# Autodesk Inventor assembly: CartesianRobotWorkSpace
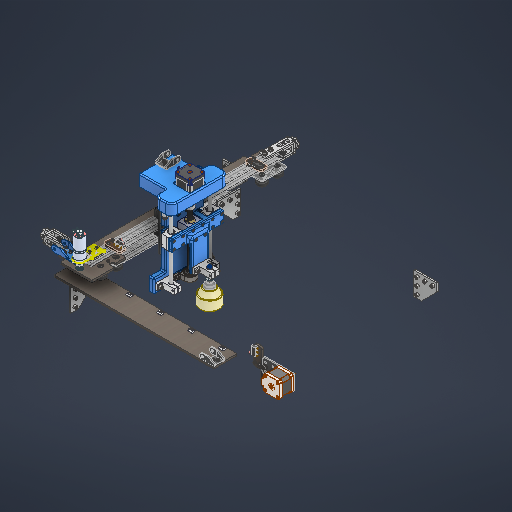
[picture p0: Inventor's stored thumbnail of the model, 512x512]
Saved by Autodesk Inventor 2027.1 (Build 311270010, 270A)
## iProperties
Created: 2026-09-29
Part Number: CartesianRobotWorkSpace
Document SubType Name: Assembly
Designer: SDS Scholar
Author: SDS Scholar
## Documents named in this file (40)
- E:\Apps\AutodeskInventor\University\MCT333_Design_of_Mechatronics_Systems_1\CAD\cartesian_robot_workspace\CartesianRobotWorkSpace.iam
- E:\Apps\AutodeskInventor\University\MCT333_Design_of_Mechatronics_Systems_1\CAD\off_the_shelf_components\AluminiumExtrusion\AluminiumExtrusion2020\Pillars.ipt
- E:\Apps\AutodeskInventor\University\MCT333_Design_of_Mechatronics_Systems_1\CAD\off_the_shelf_components\CornerBracket2020\CornerBracket2020.ipt
- E:\Apps\AutodeskInventor\University\MCT333_Design_of_Mechatronics_Systems_1\CAD\en-US\en-US\SS-ISO 4762\ISO 4762 - M5 x 10SS-ISO.ipt
- E:\Apps\AutodeskInventor\University\MCT333_Design_of_Mechatronics_Systems_1\CAD\off_the_shelf_components\T_nuts\Slider T-Nut for 2020 - M5.ipt
- E:\Apps\AutodeskInventor\University\MCT333_Design_of_Mechatronics_Systems_1\CAD\off_the_shelf_components\RightAngleCornerPlate2020\2020 corner joining plate v1.ipt
- E:\Apps\AutodeskInventor\University\MCT333_Design_of_Mechatronics_Systems_1\CAD\off_the_shelf_components\AluminiumExtrusion\Extrusion2040\2040extrusion_ipt\X_Axis.ipt
- E:\Apps\AutodeskInventor\University\MCT333_Design_of_Mechatronics_Systems_1\CAD\off_the_shelf_components\AluminiumExtrusion\AluminiumExtrusion2020\SupportBeam.ipt
- E:\Apps\AutodeskInventor\University\MCT333_Design_of_Mechatronics_Systems_1\CAD\off_the_shelf_components\VSoltGantrySetAllSizes\20mm Gantry Set\20mm Gantry Set.ipt
- E:\Apps\AutodeskInventor\University\MCT333_Design_of_Mechatronics_Systems_1\CAD\off_the_shelf_components\RightAngleCornerPlate2020\2020 corner joining plate v1_MIR2.ipt
- E:\Apps\AutodeskInventor\University\MCT333_Design_of_Mechatronics_Systems_1\CAD\off_the_shelf_components\T_nuts\Slider T-Nut for 2020 - M5_MIR2.ipt
- E:\Apps\AutodeskInventor\University\MCT333_Design_of_Mechatronics_Systems_1\CAD\off_the_shelf_components\nema-17-23-stepper-motor-mounts\NEMA 17 Flat.ipt
- E:\Apps\AutodeskInventor\University\MCT333_Design_of_Mechatronics_Systems_1\CAD\off_the_shelf_components\GT2BeltTensioner\2020 Belt Tensioner G_K.ipt
- E:\Apps\AutodeskInventor\University\MCT333_Design_of_Mechatronics_Systems_1\CAD\cartesian_robot_workspace\Y_Axis.iam
- E:\Apps\AutodeskInventor\University\MCT333_Design_of_Mechatronics_Systems_1\CAD\cartesian_robot_workspace\Z Axis\Z-Axis.iam
- E:\Apps\AutodeskInventor\University\MCT333_Design_of_Mechatronics_Systems_1\CAD\motors_and_actuators\nema17_stepper_motor\Nema17\Nema17.ipt
- E:\Apps\AutodeskInventor\University\MCT333_Design_of_Mechatronics_Systems_1\CAD\off_the_shelf_components\gt2_pulley_6\GT2 Pulley Assembly With Grub Screws\GT2 Pulley Assembly With Grub Screws.ipt
- E:\Apps\AutodeskInventor\University\MCT333_Design_of_Mechatronics_Systems_1\CAD\cartesian_robot_workspace\Z_Axis_1\Z-Axis.iam
- E:\Apps\AutodeskInventor\University\MCT333_Design_of_Mechatronics_Systems_1\CAD\cartesian_robot_workspace\LimitSwitchMountPlate.ipt
- E:\Apps\AutodeskInventor\University\MCT333_Design_of_Mechatronics_Systems_1\CAD\cartesian_robot_workspace\Z_Axis_1\NO-NC Bump Switch\NO-NC Bump Switch.ipt
- E:\Apps\AutodeskInventor\University\MCT333_Design_of_Mechatronics_Systems_1\CAD\cartesian_robot_workspace\Z_Axis_1\Slider T-Nut for 2020 - M3.ipt
- C:\Users\SDS Scholar\Documents\Inventor\Content Center Files\R2027\en-US\ISO 4762(2)\ISO 4762 - M3 x 10ISO.ipt
- C:\Users\SDS Scholar\Documents\Inventor\Content Center Files\R2027\en-US\ANSI B18.22 M\ANSI B18.22M - 3 N.ipt
- E:\Apps\AutodeskInventor\University\MCT333_Design_of_Mechatronics_Systems_1\CAD\cartesian_robot_workspace\Z_Axis_1\2020 Belt Tensioner G_K.ipt
- E:\Apps\AutodeskInventor\University\MCT333_Design_of_Mechatronics_Systems_1\CAD\cartesian_robot_workspace\Z_Axis_1\M4 T slot nut - 2020\M4 T slot nut - 2020.ipt
- C:\Users\SDS Scholar\Documents\Inventor\Content Center Files\R2027\en-US\ISO 4762(2)\ISO 4762 - M4 x 12ISO.ipt
- C:\Users\SDS Scholar\Documents\Inventor\Content Center Files\R2027\en-US\ANSI B18.22 M\ANSI B18.22M - 4 N.ipt
- E:\Apps\AutodeskInventor\University\MCT333_Design_of_Mechatronics_Systems_1\CAD\Drag Chain Support (Y Axis).ipt
- E:\Apps\AutodeskInventor\University\MCT333_Design_of_Mechatronics_Systems_1\CAD\cartesian_robot_workspace\Z_Axis_1\Drag Chain Start Link.ipt
- C:\Users\SDS Scholar\Documents\Inventor\Content Center Files\R2027\en-US\ANSI B18.22 M\ANSI B18.22M - 5 N.ipt
- C:\Users\SDS Scholar\Documents\Inventor\Content Center Files\R2027\en-US\SS-ISO 4762\ISO 4762 - M5 x 12SS-ISO.ipt
- E:\Apps\AutodeskInventor\University\MCT333_Design_of_Mechatronics_Systems_1\CAD\cartesian_robot_workspace\Z_Axis_1\LimitSwitchMountPlate (X Axis).ipt
- C:\Users\SDS Scholar\Documents\Inventor\Content Center Files\R2027\en-US\ISO 4762(2)\ISO 4762 - M3 x 12ISO.ipt
- E:\Apps\AutodeskInventor\University\MCT333_Design_of_Mechatronics_Systems_1\CAD\en-US\en-US\ISO 4762(2)\ISO 4762 - M2 x 16ISO.ipt
- E:\Apps\AutodeskInventor\University\MCT333_Design_of_Mechatronics_Systems_1\CAD\en-US\en-US\ISO 4032(2)\ISO 4032 - M2 - ISO.ipt
- E:\Apps\AutodeskInventor\University\MCT333_Design_of_Mechatronics_Systems_1\CAD\en-US\en-US\Plain Washer Metric\ANSI B18.22M - 2 N.ipt
- E:\Apps\AutodeskInventor\University\MCT333_Design_of_Mechatronics_Systems_1\CAD\en-US\en-US\ISO 7046-1 Z(1)\ISO 7045 - M2.5 x 12_ - 4.8 - Z - ISO.ipt
- E:\Apps\AutodeskInventor\University\MCT333_Design_of_Mechatronics_Systems_1\CAD\en-US\en-US\Plain Washer Metric\ANSI B18.22M - 2.5 N.ipt
- E:\Apps\AutodeskInventor\University\MCT333_Design_of_Mechatronics_Systems_1\CAD\en-US\en-US\ISO 4032(2)\ISO 4032 - M3 - ISO.ipt
- E:\Apps\AutodeskInventor\University\MCT333_Design_of_Mechatronics_Systems_1\CAD\DESIGN1_CAD_parameters.xlsx
## Components (190 placed, 36 different names)
1. Z-Axis:1 [sub-assembly] — Tangent:9, Tangent:10, Mate:231, Mate:232
2. Z-Axis:2 [sub-assembly] — Mate:299, Mate:300, Tangent:11, Flush:334, Mate:455, Mate:475
3. LimitSwitchMountPlate:1 — Mate:326, Mate:327, Mate:328, Flush:330
4. NO-NC Bump Switch:1
5. Slider T-Nut for 2020 - M3:1 — Mate:330, Angle:2, Flush:331
6. Slider T-Nut for 2020 - M3:2 — Mate:329, Angle:1, Flush:331, Mate:331
7. ISO 4762 M3 x 10:1 — Mate:327, Mate:330
8. ISO 4762 M3 x 10:2 — Mate:328, Mate:329
9. Plain Washer (Metric) 3 N:1
10. Plain Washer (Metric) 3 N:2
11. ISO 4762 M2 x 16:7
12. ISO 4032 M2:7
13. Plain Washer (Metric) 2 N:8
14. ISO 4762 M2 x 16:8
15. ISO 4032 M2:8
16. Plain Washer (Metric) 2 N:9
17. Drag Chain Start Link:1 — Mate:349, Mate:350, Mate:351, Flush:334, Mate:462, Mate:463, Mate:464, Mate:465
18. Drag Chain Support (Y Axis):1 — Mate:347, Flush:333, Mate:348, Mate:349, Mate:350, Mate:351, Mate:466, Mate:467, Mate:468, Mate:472, Mate:474
19. 2020 Belt Tensioner G_K:3 — Flush:336, Mate:382, Mate:383, Mate:455
20. M4 T slot nut - 2020:3 — Mate:384
21. M4 T slot nut - 2020:4
22. ISO 4762 M4 x 12:3
23. ISO 4762 M4 x 12:4
24. Plain Washer (Metric) 4 N:3
25. Plain Washer (Metric) 4 N:4
26. SS ISO 4762 M5 x 12:1 — Mate:385, Mate:387, Mate:393
27. SS ISO 4762 M5 x 12:2 — Mate:388, Mate:389
28. Slider T-Nut for 2020 - M5:52 — Flush:337, Flush:338, Mate:392, Angle:14
29. Slider T-Nut for 2020 - M5:53 — Flush:337, Angle:14
30. NEMA 17 Flat:2 — Mate:386, Mate:390, Mate:391, Angle:8, Angle:9, Mate:400, Mate:407, Mate:408, Mate:409, Mate:449
31. Nema17:2 — Mate:381, Angle:9, Mate:394, Mate:395, Mate:396, Mate:397
32. GT2 Pulley Assembly With Grub Screws:2 — Mate:381
33. Plain Washer (Metric) 5 N:1 — Mate:385, Mate:386, Mate:387
34. Plain Washer (Metric) 5 N:2 — Mate:388, Mate:389, Mate:390
35. ISO 7045 Z M2.5 x 12 - 4.8 - Z:6 — Mate:394, Mate:401, Mate:404
36. ISO 7045 Z M2.5 x 12 - 4.8 - Z:7 — Mate:395, Mate:398, Mate:399
37. ISO 7045 Z M2.5 x 12 - 4.8 - Z:8 — Mate:396, Mate:402, Mate:406
38. ISO 7045 Z M2.5 x 12 - 4.8 - Z:9 — Mate:397, Mate:403, Mate:405
39. Plain Washer (Metric) 2.5 N:6 — Mate:401, Mate:404, Mate:408
40. Plain Washer (Metric) 2.5 N:7 — Mate:403, Mate:405, Mate:409
41. Plain Washer (Metric) 2.5 N:8 — Mate:402, Mate:406, Mate:407
42. Plain Washer (Metric) 2.5 N:9 — Mate:398, Mate:399, Mate:400
43. Slider T-Nut for 2020 - M3:3 — Angle:12, Angle:13, Flush:339, Mate:447
44. Slider T-Nut for 2020 - M3:4 — Angle:13, Flush:339
45. ISO 4762 M3 x 10:3 — Mate:444, Mate:448
46. ISO 4762 M3 x 10:4 — Mate:443
47. Plain Washer (Metric) 3 N:3 — Mate:445
48. Plain Washer (Metric) 3 N:4 — Mate:446
49. LimitSwitchMountPlate (X Axis):1 — Angle:11, Mate:442, Mate:443, Mate:444, Mate:445, Mate:446, Angle:12, Mate:449, Mate:450, Mate:451, Mate:452, Mate:453, Mate:454, Mate:475
50. NO-NC Bump Switch:3 — Mate:452
51. ISO 4762 M2 x 16:9 — Mate:451
52. ISO 4032 M2:9 — Mate:454
53. Plain Washer (Metric) 2 N:10
54. ISO 4762 M2 x 16:10 — Mate:450
55. ISO 4032 M2:10 — Mate:453
56. Plain Washer (Metric) 2 N:11
57. ISO 4762 M3 x 12:1 — Mate:462, Mate:468
58. Plain Washer (Metric) 3 N:5 — Mate:463
59. ISO 4032 M3:3 — Mate:467
60. ISO 4762 M3 x 12:2 — Mate:464
61. Plain Washer (Metric) 3 N:6 — Mate:465
62. ISO 4032 M3:4 — Mate:466
63. SupportBeam:1 — Mate:123, Mate:124, Mate:125, Mate:126, Mate:138, Mate:141, Mate:143, Mate:202
64. X_Axis:1 — Mate:32, Mate:33, Mate:34, Mate:35, Mate:36, Mate:37, Mate:48, Mate:49, Mate:56, Mate:59, Flush:3, Tangent:1, Tangent:2, Mate:217, Mate:271, Mate:299, Tangent:11, Mate:326, Flush:330, Angle:1, Angle:2, Mate:331, Mate:347, Flush:333, Flush:336, Mate:382, Mate:383, Mate:384, Mate:391, Angle:8, Flush:338, Mate:392, Mate:393, Angle:11, Mate:442, Mate:447, Mate:448, Angle:15, Mate:473
65. X_Axis:2 — Mate:89, Mate:90, Mate:91, Mate:92, Mate:93, Mate:94, Mate:107, Mate:110, Mate:113, Mate:115, Flush:4, Tangent:5, Tangent:6, Mate:225, Mate:300
66. 2020 Belt Tensioner G_K:1 — Mate:271
67. 20mm Gantry Set:1 — Tangent:1, Tangent:2, Flush:5, Mate:171, Flush:9, Mate:229, Mate:230
68. 20mm Gantry Set:2 — Tangent:5, Tangent:6, Flush:5, Mate:174, Mate:177, Flush:8, Flush:9
69. Y_Axis:1 [sub-assembly] — Mate:167, Mate:168, Mate:169, Mate:170, Mate:173, Mate:176, Mate:177, Flush:8, Tangent:9, Tangent:10, Mate:231, Mate:232
70. Slider T-Nut for 2020 - M5:44 — Mate:167, Mate:168, Mate:172
71. Slider T-Nut for 2020 - M5:45 — Mate:169, Mate:170, Mate:175
72. SS ISO 4762 M5 x 10:62 — Mate:174, Mate:175, Mate:176
73. SS ISO 4762 M5 x 10:63 — Mate:171, Mate:172, Mate:173
74. Pillars:1 — Flush:10, Flush:11, Mate:183, Mate:184, Mate:185, Mate:186, Mate:187, Mate:188, Mate:189, Flush:191, Flush:192, Mate:190, Symmetry:1, Mate:191, Mate:192, Mate:193, Mate:194, Mate:195, Mate:196, Mate:197, Mate:198, Mate:199, Mate:200, Mate:201, Mate:202, Mate:476, Mate:477
75. SS ISO 4762 M5 x 10:2 — Mate:28, Mate:29, Mate:189
76. Slider T-Nut for 2020 - M5:2 — Mate:29, Mate:186, Mate:187
77. Slider T-Nut for 2020 - M5:1 — Mate:21, Mate:184, Mate:185
78. SS ISO 4762 M5 x 10:1 — Mate:20, Mate:21, Mate:31, Mate:188
79. CornerBracket2020:1 — Mate:20, Mate:31, Flush:191, Flush:340, Flush:341
80. CornerBracket2020:4 — Mate:28, Flush:192, Mate:190
81. CornerBracket2020:12 — Flush:341, Mate:477
82. CornerBracket2020:11 — Mate:476, Flush:340
83. Pillars:2 — Mate:218, Mate:219, Mate:220, Mate:221, Mate:222, Mate:223, Mate:224, Mate:225
84. SS ISO 4762 M5 x 10:64
85. Slider T-Nut for 2020 - M5:46
86. Slider T-Nut for 2020 - M5:47
87. SS ISO 4762 M5 x 10:65
88. CornerBracket2020:5
89. CornerBracket2020:6
90. CornerBracket2020:13
91. CornerBracket2020:14
92. Pillars:3 — Symmetry:1, Mate:348
93. SS ISO 4762 M5 x 10:66
94. Slider T-Nut for 2020 - M5:48
95. Slider T-Nut for 2020 - M5:49
96. SS ISO 4762 M5 x 10:67
97. CornerBracket2020:7
98. CornerBracket2020:8
99. CornerBracket2020:15
100. CornerBracket2020:16
101. Pillars:4 — Mate:210, Mate:211, Mate:212, Mate:213, Mate:214, Mate:215, Mate:216, Mate:217
102. SS ISO 4762 M5 x 10:68
103. Slider T-Nut for 2020 - M5:50
104. Slider T-Nut for 2020 - M5:51
105. SS ISO 4762 M5 x 10:69
106. CornerBracket2020:9
107. CornerBracket2020:10
108. CornerBracket2020:17
109. CornerBracket2020:18
110. Slider T-Nut for 2020 - M5:54 — Angle:15, Mate:473
111. Plain Washer (Metric) 5 N:3 — Mate:474
112. SS ISO 4762 M5 x 12:3 — Mate:472
113. Slider T-Nut for 2020 - M5:55
114. Plain Washer (Metric) 5 N:4
115. SS ISO 4762 M5 x 12:4
116. Slider T-Nut for 2020 - M5:56
117. Plain Washer (Metric) 5 N:5
118. SS ISO 4762 M5 x 12:5
119. Slider T-Nut for 2020 - M5:57
120. Plain Washer (Metric) 5 N:6
121. SS ISO 4762 M5 x 12:6
122. Slider T-Nut for 2020 - M5:58
123. Plain Washer (Metric) 5 N:7
124. SS ISO 4762 M5 x 12:7
125. 2020 corner joining plate v1:6 — Mate:127, Mate:130, Mate:133, Mate:136, Mate:139, Mate:143, Mate:144, Mate:201
126. Slider T-Nut for 2020 - M5:35 — Mate:131, Mate:192, Mate:195
127. Slider T-Nut for 2020 - M5:36 — Mate:123, Mate:124, Mate:137
128. Slider T-Nut for 2020 - M5:37 — Mate:134, Mate:191, Mate:194, Mate:196
129. Slider T-Nut for 2020 - M5:38 — Mate:125, Mate:126, Mate:140
130. Slider T-Nut for 2020 - M5:39 — Mate:128, Mate:193, Mate:197
131. SS ISO 4762 M5 x 10:48 — Mate:127, Mate:128, Mate:198
132. SS ISO 4762 M5 x 10:49 — Mate:139, Mate:140, Mate:141
133. SS ISO 4762 M5 x 10:50 — Mate:130, Mate:131, Mate:199
134. SS ISO 4762 M5 x 10:51 — Mate:133, Mate:134, Mate:200
135. SS ISO 4762 M5 x 10:52 — Mate:136, Mate:137, Mate:138
136. 2020 corner joining plate v1_MIR2:1
137. Slider T-Nut for 2020 - M5_MIR2:1
138. Slider T-Nut for 2020 - M5_MIR2:2
139. Slider T-Nut for 2020 - M5_MIR2:3
140. Slider T-Nut for 2020 - M5_MIR2:4
141. Slider T-Nut for 2020 - M5_MIR2:5
142. SS ISO 4762 M5 x 10:53
143. SS ISO 4762 M5 x 10:54
144. SS ISO 4762 M5 x 10:55
145. SS ISO 4762 M5 x 10:56
146. SS ISO 4762 M5 x 10:57
147. 2020 corner joining plate v1:1 — Mate:42, Mate:46, Mate:49, Mate:51, Mate:54, Mate:57, Flush:3, Mate:216, Mate:230
148. Slider T-Nut for 2020 - M5:9 — Mate:36, Mate:37, Mate:55
149. Slider T-Nut for 2020 - M5:10 — Mate:52, Mate:212, Mate:213
150. Slider T-Nut for 2020 - M5:11 — Mate:43, Mate:210, Mate:211
151. Slider T-Nut for 2020 - M5:12 — Mate:34, Mate:35, Mate:58
152. Slider T-Nut for 2020 - M5:13 — Mate:32, Mate:33, Mate:47
153. SS ISO 4762 M5 x 10:9 — Mate:42, Mate:43, Mate:215
154. SS ISO 4762 M5 x 10:10 — Mate:46, Mate:47, Mate:48
155. SS ISO 4762 M5 x 10:11 — Mate:54, Mate:55, Mate:56
156. SS ISO 4762 M5 x 10:12 — Mate:51, Mate:52, Mate:214
157. SS ISO 4762 M5 x 10:13 — Mate:57, Mate:58, Mate:59
158. 2020 corner joining plate v1:2 — Mate:229
159. Slider T-Nut for 2020 - M5:14
160. Slider T-Nut for 2020 - M5:15
161. Slider T-Nut for 2020 - M5:16
162. Slider T-Nut for 2020 - M5:17
163. Slider T-Nut for 2020 - M5:18
164. SS ISO 4762 M5 x 10:14
165. SS ISO 4762 M5 x 10:15
166. SS ISO 4762 M5 x 10:16
167. SS ISO 4762 M5 x 10:17
168. SS ISO 4762 M5 x 10:18
169. 2020 corner joining plate v1:4 — Mate:99, Mate:102, Mate:105, Mate:108, Mate:111, Mate:115, Flush:4, Mate:224
170. Slider T-Nut for 2020 - M5:25 — Mate:93, Mate:94, Mate:106
171. Slider T-Nut for 2020 - M5:26 — Mate:103, Mate:218, Mate:219
172. Slider T-Nut for 2020 - M5:27 — Mate:100, Mate:220, Mate:221
173. Slider T-Nut for 2020 - M5:28 — Mate:91, Mate:92, Mate:109
174. Slider T-Nut for 2020 - M5:29 — Mate:89, Mate:90, Mate:112
175. SS ISO 4762 M5 x 10:38 — Mate:99, Mate:100, Mate:223
176. SS ISO 4762 M5 x 10:39 — Mate:105, Mate:106, Mate:107
177. SS ISO 4762 M5 x 10:40 — Mate:102, Mate:103, Mate:222
178. SS ISO 4762 M5 x 10:41 — Mate:108, Mate:109, Mate:110
179. SS ISO 4762 M5 x 10:42 — Mate:111, Mate:112, Mate:113
180. 2020 corner joining plate v1:5 — Mate:144
181. Slider T-Nut for 2020 - M5:30
182. Slider T-Nut for 2020 - M5:31
183. Slider T-Nut for 2020 - M5:32
184. Slider T-Nut for 2020 - M5:33
185. Slider T-Nut for 2020 - M5:34
186. SS ISO 4762 M5 x 10:43
187. SS ISO 4762 M5 x 10:44
188. SS ISO 4762 M5 x 10:45
189. SS ISO 4762 M5 x 10:46
190. SS ISO 4762 M5 x 10:47
## Component patterns: (4 elements, first: Pillars:1 + SS ISO 4762 M5 x 10:2 + Slider T-Nut for 2020 - M5:2 + Slider T-Nut for 2020 - M5:1 + SS ISO 4762 M5 x 10:1 + CornerBracket2020:1 + CornerBracket2020:4 + CornerBracket2020:12 + CornerBracket2020:11), (5 elements, first: Slider T-Nut for 2020 - M5:54 + Plain Washer (Metric) 5 N:3 + SS ISO 4762 M5 x 12:3), (2 elements, first: 2020 corner joining plate v1:6 + Slider T-Nut for 2020 - M5:35 + Slider T-Nut for 2020 - M5:36 + Slider T-Nut for 2020 - M5:37 + Slider T-Nut for 2020 - M5:38 + Slider T-Nut for 2020 - M5:39 + SS ISO 4762 M5 x 10:48 + SS ISO 4762 M5 x 10:49 + SS ISO 4762 M5 x 10:50 + SS ISO 4762 M5 x 10:51 + SS ISO 4762 M5 x 10:52), (2 elements, first: 2020 corner joining plate v1:1 + Slider T-Nut for 2020 - M5:9 + Slider T-Nut for 2020 - M5:10 + Slider T-Nut for 2020 - M5:11 + Slider T-Nut for 2020 - M5:12 + Slider T-Nut for 2020 - M5:13 + SS ISO 4762 M5 x 10:9 + SS ISO 4762 M5 x 10:10 + SS ISO 4762 M5 x 10:11 + SS ISO 4762 M5 x 10:12 + SS ISO 4762 M5 x 10:13), (2 elements, first: 2020 corner joining plate v1:4 + Slider T-Nut for 2020 - M5:25 + Slider T-Nut for 2020 - M5:26 + Slider T-Nut for 2020 - M5:27 + Slider T-Nut for 2020 - M5:28 + Slider T-Nut for 2020 - M5:29 + SS ISO 4762 M5 x 10:38 + SS ISO 4762 M5 x 10:39 + SS ISO 4762 M5 x 10:40 + SS ISO 4762 M5 x 10:41 + SS ISO 4762 M5 x 10:42)
## Relationships (288: Mate 248, Flush 20, Angle 12, Tangent 7, Symmetry 1)
- Mate:20: SS ISO 4762 M5 x 10:1 ↔ CornerBracket2020:1
- Mate:21: Slider T-Nut for 2020 - M5:1 ↔ SS ISO 4762 M5 x 10:1
- Mate:28: SS ISO 4762 M5 x 10:2 ↔ CornerBracket2020:4
- Mate:29: SS ISO 4762 M5 x 10:2 ↔ Slider T-Nut for 2020 - M5:2
- Mate:31 (0.7 mm): SS ISO 4762 M5 x 10:1 ↔ CornerBracket2020:1
- Mate:32: X_Axis:1 ↔ Slider T-Nut for 2020 - M5:13
- Mate:33: X_Axis:1 ↔ Slider T-Nut for 2020 - M5:13
- Mate:34: X_Axis:1 ↔ Slider T-Nut for 2020 - M5:12
- Mate:35: X_Axis:1 ↔ Slider T-Nut for 2020 - M5:12
- Mate:36: X_Axis:1 ↔ Slider T-Nut for 2020 - M5:9
- Mate:37: X_Axis:1 ↔ Slider T-Nut for 2020 - M5:9
- Mate:42: 2020 corner joining plate v1:1 ↔ SS ISO 4762 M5 x 10:9
- Mate:43: Slider T-Nut for 2020 - M5:11 ↔ SS ISO 4762 M5 x 10:9
- Mate:46: 2020 corner joining plate v1:1 ↔ SS ISO 4762 M5 x 10:10
- Mate:47: Slider T-Nut for 2020 - M5:13 ↔ SS ISO 4762 M5 x 10:10
- Mate:48: X_Axis:1 ↔ SS ISO 4762 M5 x 10:10
- Mate:49: X_Axis:1 ↔ 2020 corner joining plate v1:1
- Mate:51: 2020 corner joining plate v1:1 ↔ SS ISO 4762 M5 x 10:12
- Mate:52: Slider T-Nut for 2020 - M5:10 ↔ SS ISO 4762 M5 x 10:12
- Mate:54: 2020 corner joining plate v1:1 ↔ SS ISO 4762 M5 x 10:11
- Mate:55: Slider T-Nut for 2020 - M5:9 ↔ SS ISO 4762 M5 x 10:11
- Mate:56: X_Axis:1 ↔ SS ISO 4762 M5 x 10:11
- Mate:57: 2020 corner joining plate v1:1 ↔ SS ISO 4762 M5 x 10:13
- Mate:58: Slider T-Nut for 2020 - M5:12 ↔ SS ISO 4762 M5 x 10:13
- Mate:59: X_Axis:1 ↔ SS ISO 4762 M5 x 10:13
- Flush:3: X_Axis:1 ↔ 2020 corner joining plate v1:1
- Tangent:1: X_Axis:1 ↔ 20mm Gantry Set:1
- Tangent:2: X_Axis:1 ↔ 20mm Gantry Set:1
- Mate:89: X_Axis:2 ↔ Slider T-Nut for 2020 - M5:29
- Mate:90: X_Axis:2 ↔ Slider T-Nut for 2020 - M5:29
- Mate:91: X_Axis:2 ↔ Slider T-Nut for 2020 - M5:28
- Mate:92: X_Axis:2 ↔ Slider T-Nut for 2020 - M5:28
- Mate:93: X_Axis:2 ↔ Slider T-Nut for 2020 - M5:25
- Mate:94: X_Axis:2 ↔ Slider T-Nut for 2020 - M5:25
- Mate:99: 2020 corner joining plate v1:4 ↔ SS ISO 4762 M5 x 10:38
- Mate:100: Slider T-Nut for 2020 - M5:27 ↔ SS ISO 4762 M5 x 10:38
- Mate:102: 2020 corner joining plate v1:4 ↔ SS ISO 4762 M5 x 10:40
- Mate:103: Slider T-Nut for 2020 - M5:26 ↔ SS ISO 4762 M5 x 10:40
- Mate:105: 2020 corner joining plate v1:4 ↔ SS ISO 4762 M5 x 10:39
- Mate:106: Slider T-Nut for 2020 - M5:25 ↔ SS ISO 4762 M5 x 10:39
- Mate:107: X_Axis:2 ↔ SS ISO 4762 M5 x 10:39
- Mate:108: 2020 corner joining plate v1:4 ↔ SS ISO 4762 M5 x 10:41
- Mate:109: Slider T-Nut for 2020 - M5:28 ↔ SS ISO 4762 M5 x 10:41
- Mate:110: X_Axis:2 ↔ SS ISO 4762 M5 x 10:41
- Mate:111: 2020 corner joining plate v1:4 ↔ SS ISO 4762 M5 x 10:42
- Mate:112: Slider T-Nut for 2020 - M5:29 ↔ SS ISO 4762 M5 x 10:42
- Mate:113: X_Axis:2 ↔ SS ISO 4762 M5 x 10:42
- Mate:115: X_Axis:2 ↔ 2020 corner joining plate v1:4
- Flush:4: X_Axis:2 ↔ 2020 corner joining plate v1:4
- Mate:123: SupportBeam:1 ↔ Slider T-Nut for 2020 - M5:36
- Mate:124: SupportBeam:1 ↔ Slider T-Nut for 2020 - M5:36
- Mate:125: SupportBeam:1 ↔ Slider T-Nut for 2020 - M5:38
- Mate:126: SupportBeam:1 ↔ Slider T-Nut for 2020 - M5:38
- Mate:127: 2020 corner joining plate v1:6 ↔ SS ISO 4762 M5 x 10:48
- Mate:128: Slider T-Nut for 2020 - M5:39 ↔ SS ISO 4762 M5 x 10:48
- Mate:130: 2020 corner joining plate v1:6 ↔ SS ISO 4762 M5 x 10:50
- Mate:131: Slider T-Nut for 2020 - M5:35 ↔ SS ISO 4762 M5 x 10:50
- Mate:133: 2020 corner joining plate v1:6 ↔ SS ISO 4762 M5 x 10:51
- Mate:134: Slider T-Nut for 2020 - M5:37 ↔ SS ISO 4762 M5 x 10:51
- Mate:136: 2020 corner joining plate v1:6 ↔ SS ISO 4762 M5 x 10:52
- Mate:137: Slider T-Nut for 2020 - M5:36 ↔ SS ISO 4762 M5 x 10:52
- Mate:138: SupportBeam:1 ↔ SS ISO 4762 M5 x 10:52
- Mate:139: 2020 corner joining plate v1:6 ↔ SS ISO 4762 M5 x 10:49
- Mate:140: Slider T-Nut for 2020 - M5:38 ↔ SS ISO 4762 M5 x 10:49
- Mate:141: SupportBeam:1 ↔ SS ISO 4762 M5 x 10:49
- Mate:143: SupportBeam:1 ↔ 2020 corner joining plate v1:6
- Mate:144 (5 mm): 2020 corner joining plate v1:6 ↔ 2020 corner joining plate v1:5
- Tangent:5: X_Axis:2 ↔ 20mm Gantry Set:2
- Tangent:6: X_Axis:2 ↔ 20mm Gantry Set:2
- Flush:5: 20mm Gantry Set:1 ↔ 20mm Gantry Set:2
- Mate:167: Y_Axis:1 ↔ Slider T-Nut for 2020 - M5:44
- Mate:168: Y_Axis:1 ↔ Slider T-Nut for 2020 - M5:44
- Mate:169: Y_Axis:1 ↔ Slider T-Nut for 2020 - M5:45
- Mate:170: Y_Axis:1 ↔ Slider T-Nut for 2020 - M5:45
- Mate:171: 20mm Gantry Set:1 ↔ SS ISO 4762 M5 x 10:63
- Mate:172: Slider T-Nut for 2020 - M5:44 ↔ SS ISO 4762 M5 x 10:63
- Mate:173: Y_Axis:1 ↔ SS ISO 4762 M5 x 10:63
- Mate:174: 20mm Gantry Set:2 ↔ SS ISO 4762 M5 x 10:62
- Mate:175: Slider T-Nut for 2020 - M5:45 ↔ SS ISO 4762 M5 x 10:62
- Mate:176: Y_Axis:1 ↔ SS ISO 4762 M5 x 10:62
- Mate:177: 20mm Gantry Set:2 ↔ Y_Axis:1
- Flush:8 (-20 mm): 20mm Gantry Set:2 ↔ Y_Axis:1
- Flush:9: 20mm Gantry Set:1 ↔ 20mm Gantry Set:2
- Flush:10: Pillars:1
- Flush:11: Pillars:1
- Mate:183: Pillars:1
- Mate:184: Pillars:1 ↔ Slider T-Nut for 2020 - M5:1
- Mate:185: Pillars:1 ↔ Slider T-Nut for 2020 - M5:1
- Mate:186: Pillars:1 ↔ Slider T-Nut for 2020 - M5:2
- Mate:187: Pillars:1 ↔ Slider T-Nut for 2020 - M5:2
- Mate:188: Pillars:1 ↔ SS ISO 4762 M5 x 10:1
- Mate:189: Pillars:1 ↔ SS ISO 4762 M5 x 10:2
- Flush:191 (63 mm): Pillars:1 ↔ CornerBracket2020:1
- Flush:192 (63 mm): Pillars:1 ↔ CornerBracket2020:4
- Mate:190: Pillars:1 ↔ CornerBracket2020:4
- Symmetry:1: Pillars:1 ↔ Pillars:3
- Mate:191: Pillars:1 ↔ Slider T-Nut for 2020 - M5:37
- Mate:192: Pillars:1 ↔ Slider T-Nut for 2020 - M5:35
- Mate:193: Pillars:1 ↔ Slider T-Nut for 2020 - M5:39
- Mate:194: Pillars:1 ↔ Slider T-Nut for 2020 - M5:37
- Mate:195: Pillars:1 ↔ Slider T-Nut for 2020 - M5:35
- Mate:196: Pillars:1 ↔ Slider T-Nut for 2020 - M5:37
- Mate:197: Pillars:1 ↔ Slider T-Nut for 2020 - M5:39
- Mate:198: Pillars:1 ↔ SS ISO 4762 M5 x 10:48
- Mate:199: Pillars:1 ↔ SS ISO 4762 M5 x 10:50
- Mate:200: Pillars:1 ↔ SS ISO 4762 M5 x 10:51
- Mate:201: Pillars:1 ↔ 2020 corner joining plate v1:6
- Mate:202: SupportBeam:1 ↔ Pillars:1
- Mate:210: Pillars:4 ↔ Slider T-Nut for 2020 - M5:11
- Mate:211: Pillars:4 ↔ Slider T-Nut for 2020 - M5:11
- Mate:212: Pillars:4 ↔ Slider T-Nut for 2020 - M5:10
- Mate:213: Pillars:4 ↔ Slider T-Nut for 2020 - M5:10
- Mate:214: Pillars:4 ↔ SS ISO 4762 M5 x 10:12
- Mate:215: Pillars:4 ↔ SS ISO 4762 M5 x 10:9
- Mate:216: Pillars:4 ↔ 2020 corner joining plate v1:1
- Mate:217: X_Axis:1 ↔ Pillars:4
- Mate:218: Pillars:2 ↔ Slider T-Nut for 2020 - M5:26
- Mate:219: Pillars:2 ↔ Slider T-Nut for 2020 - M5:26
- Mate:220: Pillars:2 ↔ Slider T-Nut for 2020 - M5:27
- Mate:221: Pillars:2 ↔ Slider T-Nut for 2020 - M5:27
- Mate:222: Pillars:2 ↔ SS ISO 4762 M5 x 10:40
- Mate:223: Pillars:2 ↔ SS ISO 4762 M5 x 10:38
- Mate:224: Pillars:2 ↔ 2020 corner joining plate v1:4
- Mate:225: X_Axis:2 ↔ Pillars:2
- Tangent:9: Z-Axis:1 ↔ Y_Axis:1
- Tangent:10: Z-Axis:1 ↔ Y_Axis:1
- Mate:229: 20mm Gantry Set:1 ↔ 2020 corner joining plate v1:2
- Mate:230: 20mm Gantry Set:1 ↔ 2020 corner joining plate v1:1
- Mate:231: Z-Axis:1 ↔ Y_Axis:1
- Mate:232: Z-Axis:1 ↔ Y_Axis:1
- Mate:271: X_Axis:1 ↔ 2020 Belt Tensioner G_K:1
- Mate:299 (3.395 mm): Z-Axis:2 ↔ X_Axis:1
- Mate:300 (3.395 mm): Z-Axis:2 ↔ X_Axis:2
- Tangent:11: Z-Axis:2 ↔ X_Axis:1
- [Mate]: LimitSwitchMountPlate:1 ↔ NO-NC Bump Switch:1
- [Mate]: LimitSwitchMountPlate:1 ↔ NO-NC Bump Switch:1
- [Mate]: LimitSwitchMountPlate:1 ↔ NO-NC Bump Switch:1
- [Mate]: ISO 4762 M3 x 10:1 ↔ Plain Washer (Metric) 3 N:1
- [Mate]: ISO 4762 M3 x 10:1 ↔ Plain Washer (Metric) 3 N:1
- [Mate]: ISO 4762 M3 x 10:2 ↔ Plain Washer (Metric) 3 N:2
- [Mate]: ISO 4762 M3 x 10:2 ↔ Plain Washer (Metric) 3 N:2
- [Mate]: LimitSwitchMountPlate:1 ↔ Plain Washer (Metric) 3 N:1
- [Mate]: LimitSwitchMountPlate:1 ↔ Plain Washer (Metric) 3 N:2
- [Mate]: ISO 4762 M2 x 16:7 ↔ ISO 4032 M2:7
- [Mate]: ISO 4762 M2 x 16:7 ↔ Plain Washer (Metric) 2 N:8
- [Mate]: ISO 4762 M2 x 16:7 ↔ Plain Washer (Metric) 2 N:8
- [Mate]: ISO 4762 M2 x 16:8 ↔ ISO 4032 M2:8
- [Mate]: ISO 4762 M2 x 16:8 ↔ Plain Washer (Metric) 2 N:9
- [Mate]: ISO 4762 M2 x 16:8 ↔ Plain Washer (Metric) 2 N:9
- [Mate]: NO-NC Bump Switch:1 ↔ ISO 4762 M2 x 16:7
- [Mate]: NO-NC Bump Switch:1 ↔ ISO 4762 M2 x 16:8
- [Mate]: NO-NC Bump Switch:1 ↔ Plain Washer (Metric) 2 N:8
- [Mate]: NO-NC Bump Switch:1 ↔ Plain Washer (Metric) 2 N:9
- [Mate]: LimitSwitchMountPlate:1 ↔ ISO 4032 M2:8
- [Mate]: LimitSwitchMountPlate:1 ↔ ISO 4032 M2:7
- Mate:326: LimitSwitchMountPlate:1 ↔ X_Axis:1
- Mate:327: LimitSwitchMountPlate:1 ↔ ISO 4762 M3 x 10:1
- Mate:328: LimitSwitchMountPlate:1 ↔ ISO 4762 M3 x 10:2
- Flush:330: LimitSwitchMountPlate:1 ↔ X_Axis:1
- Mate:329: Slider T-Nut for 2020 - M3:2 ↔ ISO 4762 M3 x 10:2
- Mate:330: Slider T-Nut for 2020 - M3:1 ↔ ISO 4762 M3 x 10:1
- Angle:1 (0 deg): Slider T-Nut for 2020 - M3:2 ↔ X_Axis:1
- Angle:2 (0 deg): Slider T-Nut for 2020 - M3:1 ↔ X_Axis:1
- Flush:331: Slider T-Nut for 2020 - M3:1 ↔ Slider T-Nut for 2020 - M3:2
- Mate:331: Slider T-Nut for 2020 - M3:2 ↔ X_Axis:1
- Mate:347: Drag Chain Support (Y Axis):1 ↔ X_Axis:1
- Flush:333: Drag Chain Support (Y Axis):1 ↔ X_Axis:1
- Mate:348 (1 mm): Drag Chain Support (Y Axis):1 ↔ Pillars:3
- Mate:349: Drag Chain Start Link:1 ↔ Drag Chain Support (Y Axis):1
- Mate:350 (2 mm): Drag Chain Start Link:1 ↔ Drag Chain Support (Y Axis):1
- Mate:351 (2 mm): Drag Chain Start Link:1 ↔ Drag Chain Support (Y Axis):1
- Flush:334: Z-Axis:2 ↔ Drag Chain Start Link:1
- [Mate]: 2020 Belt Tensioner G_K:3 ↔ M4 T slot nut - 2020:3
- [Mate]: 2020 Belt Tensioner G_K:3 ↔ M4 T slot nut - 2020:4
- [Angle] (90 deg): 2020 Belt Tensioner G_K:3 ↔ M4 T slot nut - 2020:4
- [Mate]: 2020 Belt Tensioner G_K:3 ↔ ISO 4762 M4 x 12:3
- [Mate]: 2020 Belt Tensioner G_K:3 ↔ ISO 4762 M4 x 12:4
- [Mate]: ISO 4762 M4 x 12:3 ↔ Plain Washer (Metric) 4 N:3
- [Mate]: ISO 4762 M4 x 12:4 ↔ Plain Washer (Metric) 4 N:4
- [Mate]: 2020 Belt Tensioner G_K:3 ↔ Plain Washer (Metric) 4 N:3
- [Mate]: 2020 Belt Tensioner G_K:3 ↔ Plain Washer (Metric) 4 N:4
- [Mate]: ISO 4762 M4 x 12:4 ↔ Plain Washer (Metric) 4 N:4
- [Mate]: ISO 4762 M4 x 12:3 ↔ Plain Washer (Metric) 4 N:3
- [Flush]: M4 T slot nut - 2020:3 ↔ M4 T slot nut - 2020:4
- [Angle] (0 deg): M4 T slot nut - 2020:3 ↔ M4 T slot nut - 2020:4
- [Mate]: SS ISO 4762 M5 x 12:2 ↔ Slider T-Nut for 2020 - M5:52
- [Mate]: SS ISO 4762 M5 x 12:1 ↔ Slider T-Nut for 2020 - M5:53
- [Mate]: SS ISO 4762 M5 x 12:2 ↔ Slider T-Nut for 2020 - M5:52
- [Mate]: SS ISO 4762 M5 x 12:1 ↔ NEMA 17 Flat:2
- [Mate]: SS ISO 4762 M5 x 12:2 ↔ NEMA 17 Flat:2
- [Mate]: NEMA 17 Flat:2 ↔ Nema17:2
- [Mate]: NEMA 17 Flat:2 ↔ Nema17:2
- [Mate]: Nema17:2 ↔ GT2 Pulley Assembly With Grub Screws:2
- Mate:381 (0.5 mm): Nema17:2 ↔ GT2 Pulley Assembly With Grub Screws:2
- Flush:336: 2020 Belt Tensioner G_K:3 ↔ X_Axis:1
- Mate:382: 2020 Belt Tensioner G_K:3 ↔ X_Axis:1
- Mate:383 (2 mm): 2020 Belt Tensioner G_K:3 ↔ X_Axis:1
- Mate:384: M4 T slot nut - 2020:3 ↔ X_Axis:1
- Mate:385: SS ISO 4762 M5 x 12:1 ↔ Plain Washer (Metric) 5 N:1
- Mate:386: NEMA 17 Flat:2 ↔ Plain Washer (Metric) 5 N:1
- Mate:387: SS ISO 4762 M5 x 12:1 ↔ Plain Washer (Metric) 5 N:1
- Flush:337: Slider T-Nut for 2020 - M5:52 ↔ Slider T-Nut for 2020 - M5:53
- Mate:388: SS ISO 4762 M5 x 12:2 ↔ Plain Washer (Metric) 5 N:2
- Mate:389: SS ISO 4762 M5 x 12:2 ↔ Plain Washer (Metric) 5 N:2
- Mate:390: NEMA 17 Flat:2 ↔ Plain Washer (Metric) 5 N:2
- Mate:391: NEMA 17 Flat:2 ↔ X_Axis:1
- Angle:8 (0 deg): NEMA 17 Flat:2 ↔ X_Axis:1
- Angle:9 (270 deg): NEMA 17 Flat:2 ↔ Nema17:2
- Flush:338: Slider T-Nut for 2020 - M5:52 ↔ X_Axis:1
- Mate:392: Slider T-Nut for 2020 - M5:52 ↔ X_Axis:1
- Mate:393 (3.395 mm): SS ISO 4762 M5 x 12:1 ↔ X_Axis:1
- Mate:394: Nema17:2 ↔ ISO 7045 Z M2.5 x 12 - 4.8 - Z:6
- Mate:395: Nema17:2 ↔ ISO 7045 Z M2.5 x 12 - 4.8 - Z:7
- Mate:396: Nema17:2 ↔ ISO 7045 Z M2.5 x 12 - 4.8 - Z:8
- Mate:397: Nema17:2 ↔ ISO 7045 Z M2.5 x 12 - 4.8 - Z:9
- Mate:398: ISO 7045 Z M2.5 x 12 - 4.8 - Z:7 ↔ Plain Washer (Metric) 2.5 N:9
- Mate:399: ISO 7045 Z M2.5 x 12 - 4.8 - Z:7 ↔ Plain Washer (Metric) 2.5 N:9
- Mate:400: NEMA 17 Flat:2 ↔ Plain Washer (Metric) 2.5 N:9
- Mate:401: ISO 7045 Z M2.5 x 12 - 4.8 - Z:6 ↔ Plain Washer (Metric) 2.5 N:6
- Mate:402: ISO 7045 Z M2.5 x 12 - 4.8 - Z:8 ↔ Plain Washer (Metric) 2.5 N:8
- Mate:403: ISO 7045 Z M2.5 x 12 - 4.8 - Z:9 ↔ Plain Washer (Metric) 2.5 N:7
- Mate:404: ISO 7045 Z M2.5 x 12 - 4.8 - Z:6 ↔ Plain Washer (Metric) 2.5 N:6
- Mate:405: ISO 7045 Z M2.5 x 12 - 4.8 - Z:9 ↔ Plain Washer (Metric) 2.5 N:7
- Mate:406: ISO 7045 Z M2.5 x 12 - 4.8 - Z:8 ↔ Plain Washer (Metric) 2.5 N:8
- Mate:407: NEMA 17 Flat:2 ↔ Plain Washer (Metric) 2.5 N:8
- Mate:408: NEMA 17 Flat:2 ↔ Plain Washer (Metric) 2.5 N:6
- Mate:409: NEMA 17 Flat:2 ↔ Plain Washer (Metric) 2.5 N:7
- [Angle] (0 deg): Slider T-Nut for 2020 - M3:3 ↔ Slider T-Nut for 2020 - M3:4
- [Mate]: ISO 4762 M3 x 10:3 ↔ Plain Washer (Metric) 3 N:3
- [Mate]: ISO 4762 M3 x 10:3 ↔ Plain Washer (Metric) 3 N:3
- [Mate]: ISO 4762 M3 x 10:4 ↔ Plain Washer (Metric) 3 N:4
- [Mate]: ISO 4762 M3 x 10:4 ↔ Plain Washer (Metric) 3 N:4
- [Mate]: Slider T-Nut for 2020 - M3:4 ↔ ISO 4762 M3 x 10:3
- [Mate]: Slider T-Nut for 2020 - M3:3 ↔ ISO 4762 M3 x 10:4
- [Mate]: ISO 4762 M2 x 16:9 ↔ ISO 4032 M2:9
- [Mate]: ISO 4762 M2 x 16:9 ↔ Plain Washer (Metric) 2 N:10
- [Mate]: ISO 4762 M2 x 16:9 ↔ Plain Washer (Metric) 2 N:10
- [Mate]: ISO 4762 M2 x 16:10 ↔ ISO 4032 M2:10
- [Mate]: ISO 4762 M2 x 16:10 ↔ Plain Washer (Metric) 2 N:11
- [Mate]: ISO 4762 M2 x 16:10 ↔ Plain Washer (Metric) 2 N:11
- [Mate]: NO-NC Bump Switch:3 ↔ ISO 4762 M2 x 16:9
- [Mate]: NO-NC Bump Switch:3 ↔ ISO 4762 M2 x 16:10
- [Mate]: NO-NC Bump Switch:3 ↔ Plain Washer (Metric) 2 N:10
- [Mate]: NO-NC Bump Switch:3 ↔ Plain Washer (Metric) 2 N:11
- Angle:11 (0 deg): LimitSwitchMountPlate (X Axis):1 ↔ X_Axis:1
- Mate:442: LimitSwitchMountPlate (X Axis):1 ↔ X_Axis:1
- Mate:443: ISO 4762 M3 x 10:4 ↔ LimitSwitchMountPlate (X Axis):1
- Mate:444: ISO 4762 M3 x 10:3 ↔ LimitSwitchMountPlate (X Axis):1
- Mate:445: Plain Washer (Metric) 3 N:3 ↔ LimitSwitchMountPlate (X Axis):1
- Mate:446: Plain Washer (Metric) 3 N:4 ↔ LimitSwitchMountPlate (X Axis):1
- Angle:12 (0 deg): Slider T-Nut for 2020 - M3:3 ↔ LimitSwitchMountPlate (X Axis):1
- Angle:13 (0 deg): Slider T-Nut for 2020 - M3:3 ↔ Slider T-Nut for 2020 - M3:4
- Flush:339: Slider T-Nut for 2020 - M3:3 ↔ Slider T-Nut for 2020 - M3:4
- Mate:447: Slider T-Nut for 2020 - M3:3 ↔ X_Axis:1
- Mate:448 (3.395 mm): ISO 4762 M3 x 10:3 ↔ X_Axis:1
- Mate:449 (2 mm): NEMA 17 Flat:2 ↔ LimitSwitchMountPlate (X Axis):1
- Mate:450: LimitSwitchMountPlate (X Axis):1 ↔ ISO 4762 M2 x 16:10
- Mate:451: LimitSwitchMountPlate (X Axis):1 ↔ ISO 4762 M2 x 16:9
- Mate:452: LimitSwitchMountPlate (X Axis):1 ↔ NO-NC Bump Switch:3
- Mate:453: LimitSwitchMountPlate (X Axis):1 ↔ ISO 4032 M2:10
- Mate:454: LimitSwitchMountPlate (X Axis):1 ↔ ISO 4032 M2:9
- Mate:455: Z-Axis:2 ↔ 2020 Belt Tensioner G_K:3
- [Mate]: ISO 4762 M3 x 12:1 ↔ Plain Washer (Metric) 3 N:5
- [Mate]: ISO 4762 M3 x 12:1 ↔ Plain Washer (Metric) 3 N:5
- [Mate]: ISO 4762 M3 x 12:1 ↔ ISO 4032 M3:3
- [Mate]: ISO 4762 M3 x 12:2 ↔ Plain Washer (Metric) 3 N:6
- [Mate]: ISO 4762 M3 x 12:2 ↔ Plain Washer (Metric) 3 N:6
- [Mate]: ISO 4762 M3 x 12:2 ↔ ISO 4032 M3:4
- Mate:462 (2 mm): Drag Chain Start Link:1 ↔ ISO 4762 M3 x 12:1
- Mate:463: Drag Chain Start Link:1 ↔ Plain Washer (Metric) 3 N:5
- Mate:464 (2 mm): Drag Chain Start Link:1 ↔ ISO 4762 M3 x 12:2
- Mate:465: Drag Chain Start Link:1 ↔ Plain Washer (Metric) 3 N:6
- Mate:466: Drag Chain Support (Y Axis):1 ↔ ISO 4032 M3:4
- Mate:467: Drag Chain Support (Y Axis):1 ↔ ISO 4032 M3:3
- Mate:468: Drag Chain Support (Y Axis):1 ↔ ISO 4762 M3 x 12:1
- Angle:14 (0 deg): Slider T-Nut for 2020 - M5:52 ↔ Slider T-Nut for 2020 - M5:53
- [Mate]: Slider T-Nut for 2020 - M5:54 ↔ SS ISO 4762 M5 x 12:3
- [Mate]: Plain Washer (Metric) 5 N:3 ↔ SS ISO 4762 M5 x 12:3
- [Mate]: Plain Washer (Metric) 5 N:3 ↔ SS ISO 4762 M5 x 12:3
- Mate:472: Drag Chain Support (Y Axis):1 ↔ SS ISO 4762 M5 x 12:3
- Angle:15 (0 deg): X_Axis:1 ↔ Slider T-Nut for 2020 - M5:54
- Mate:473: X_Axis:1 ↔ Slider T-Nut for 2020 - M5:54
- Mate:474: Drag Chain Support (Y Axis):1 ↔ Plain Washer (Metric) 5 N:3
- Mate:475: Z-Axis:2 ↔ LimitSwitchMountPlate (X Axis):1
- Mate:476: Pillars:1 ↔ CornerBracket2020:11
- Flush:340: CornerBracket2020:1 ↔ CornerBracket2020:11
- Flush:341: CornerBracket2020:1 ↔ CornerBracket2020:12
- Mate:477: Pillars:1 ↔ CornerBracket2020:12
## Named parameters: Product_dia = 50 mm, ProductBaseHeight = 40 mm, ProductLedHeight = 20 mm, GridProcutClearance = 5 mm, GridBorderThickness = 5 mm, GridBorderFillets = 7 mm, GridTotalSize = 65 mm, GridRobotClearance = 65 mm, AluminiumExtrusionBase = 20 mm, AluminiumExtrusionClearance = 35 mm, BaseTotalWidth = 680 mm, FeedingAreaLength = 340 mm, BaseTotalLength = 885 mm, DistanceBetweenGrid = 10 mm, WorkspaceLength = 515 mm, WorkspaceWidth = 440 mm, WorkspaceHeight = 183 mm, AxesBaseFillet = 15 mm, Zaxis = 197 mm, ProductTotalHeight = 45 mm, VerticalClearance = 20 mm, VerticalStroke = 105 mm, FrontArea = 50 mm, BackArea = 165 mm, CylinderStroke = 75 mm, SideAreaWidth = 200 mm, BaseHeight = 70 mm, ContolBoxLength = 100 mm, DistanceBetweenBoxes = 30 mm, BoxesWidth = 125 mm, PowerBoxLength = 660 mm, PneumaticBoxLength = 200 mm, BoxesClearance = 40 mm, BoxesHeight = 80 mm, ContolBoxWidth = 200 mm, ControlBoxHeight = 70 mm, BaseWoodThickness = 7 mm, kerf = 1.5 mm, Kerf = 0.3 mm, TransmitterAreaWidth = 100 mm, RxThickness = 1.8 mm, d738_d558_d544_d315 = 0 mm, d739_d559_d545_d168 = 0 mm, d740_d563 = 0 mm, d741_d558_d544_d315 = 0 mm, d742_d559_d545_d168 = 0 mm, d743_d563 = 0 mm, d812_d744 = 0 mm, d813_d745 = 0 mm, d814_d746 = 0 mm, d815_d747 = 0 mm, d816_d748 = 0 mm, d817_d749 = 0 mm, d724_d585 = 0 mm, d725_d587 = 0 mm, d726_d589 = 0 mm, d727_d591 = 0 mm, d823_d669 = 0 mm, d824_d670 = 0 mm, d825_d671 = 0 mm, d894_d703 = 0 mm, d895_d704 = 0 mm, d896_d706 = 90 deg, d897_d711 = 0 mm, d898_d712 = 0 mm, d899_d842_d717 = 0 mm, d900_d843_d718 = 0 mm, d901_d719 = 0 mm, d902_d720 = 0 mm, d903_d846_d721 = 0 mm, d904_d722 = 0 mm, d905_d848 = 0 mm, d906_d849 = 0 deg, d913_d755 = 0 mm, d914_d756 = 0 mm, d915_d757 = 0.5 mm, d916_d716 = 0 mm, d917_d717 = 0 mm, d918_d743 = 0 mm, d924_d572 = 0 mm, d925_d575 = 0 mm, d926_d594 = 0 mm, d723_d582 = 0 deg, d1031_d724_d585 = 0 mm, d1032_d725_d587 = 0 mm, d1033_d726_d589 = 0 mm, d1034_d727_d591 = 0 mm, d1045_d1020_d738_d558_d544_d315 = 0 mm, d1046_d1021_d739_d559_d545_d168 = 0 mm, d1047_d1022_d740_d563 = 0 mm, d1048_d1023_d741_d558_d544_d315 = 0 mm, d1049_d1024_d742_d559_d545_d168 = 0 mm, d1050_d1025_d743_d563 = 0 mm, d1051_d744 = 0 mm, d1052_d745 = 0 mm, d1053_d746 = 0 mm, d1054_d747 = 0 mm, d888_d866_d863 = 0 mm, d889_d867_d842_d688_d544_d315 = 0 mm, d890_d868_d844_d690_d566 = 0 mm, d891_d872_d863 = 0 mm, d892_d873_d842_d688_d544_d315 = 0 mm, d893_d874_d844_d690_d566 = 0 mm, d1090_d931 = 0 mm, d1091_d933 = 0 mm, d1092_d925_d575 = 0 mm, support_2 = 265 mm, support_1 = 160 mm, wood_log = 50 mm
